# Autodesk Inventor assembly: Ensamble_general
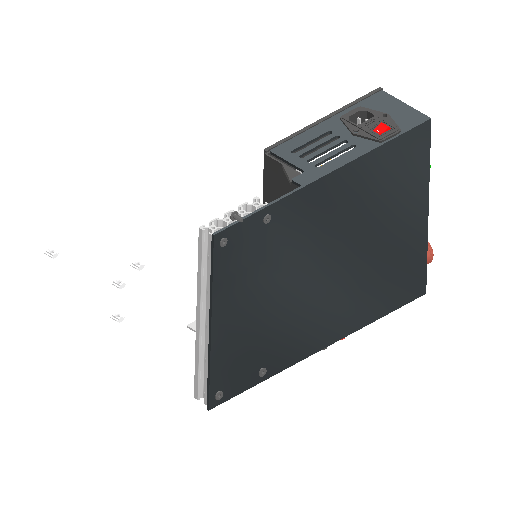
[picture p0: Inventor's stored thumbnail of the model, 512x512]
Saved by Autodesk Inventor 2025 (Build 290162000, 162)
## iProperties
Created: 2026-01-23
Part Number: Ensamble_general
Document SubType Name: Assembly
Designer: HP
Author: HP
## Documents named in this file (15)
- C:\Users\HP\Desktop\CAD\Ensamble_general.iam
- C:\Users\HP\Desktop\CAD\Chasis\Chasis_CONTROL.ipt
- C:\Users\HP\Desktop\CAD\AC_INTERUP\AC_INTERUP.ipt
- C:\Users\HP\Desktop\CAD\Banana Socket (Red)\Banana Socket (Red).ipt
- C:\Users\HP\Desktop\CAD\Banana Socket (Black)\Banana Socket (Black).ipt
- C:\Users\HP\Desktop\CAD\RED LED BULB_F\RED LED BULB_F.ipt
- C:\Users\HP\Desktop\CAD\GREEN LED BULB_F\GREEN LED BULB_F.ipt
- C:\Users\HP\Desktop\CAD\Profiles\Profiles.ipt
- C:\Users\HP\Desktop\CAD\Fuente-switching\Fuente-switching.iam
- C:\Users\HP\Desktop\CAD\E-Stop\E-Stop.ipt
- C:\Users\HP\Desktop\CAD\Tapa_chasis.ipt
- C:\Users\HP\Desktop\CAD\BRACKET_MOTOR.ipt
- C:\Users\HP\Desktop\CAD\DC Planetary Gear Brush Motor (PZ22GR9120R-084BBH)\DC Planetary Gear Brush Motor (PZ22GR9120R-084BBH).ipt
- C:\Users\HP\Desktop\CAD\Slider T-Nut for 2020 - M5\Slider T-Nut for 2020 - M5.ipt
- C:\Users\HP\Desktop\CAD\TORNILLO ALLEN CABEZA PLANA M3x0.5x6\TORNILLO ALLEN CABEZA PLANA M5x0.5x6.ipt
## Components (35 placed, 14 different names)
1. Chasis_CONTROL:1 — Coincidencia:1, Coincidencia:2, Coincidencia:3, Coincidencia:4, Coincidencia:5, Coincidencia:6, Coincidencia:7, Coincidencia:9, Coincidencia:10, Coincidencia:11, Coincidencia:12, Nivelación:1, Coincidencia:14, Nivelación:2, Coincidencia:15, Coincidencia:16, Nivelación:3, Coincidencia:19, Coincidencia:20, Coincidencia:21, Coincidencia:22, Coincidencia:23, Coincidencia:34, Coincidencia:37, Coincidencia:39, Coincidencia:41, Coincidencia:50, Coincidencia:51, Coincidencia:52, Coincidencia:53, Coincidencia:54, Coincidencia:55, Coincidencia:56, Coincidencia:57
2. AC_INTERUP:1 — Coincidencia:1, Coincidencia:2, Coincidencia:3
3. Banana Socket (Red):1 — Coincidencia:4, Coincidencia:5
4. Banana Socket (Black):1 — Coincidencia:6, Coincidencia:7
5. RED LED BULB_F:1 — Coincidencia:9, Coincidencia:12
6. GREEN LED BULB_F:1 — Coincidencia:10, Coincidencia:11
7. Profiles:1 — Nivelación:1, Coincidencia:14, Nivelación:2, Nivelación:5, Coincidencia:28, Nivelación:6, Coincidencia:32, Coincidencia:33, Coincidencia:36, Coincidencia:38, Coincidencia:40, Coincidencia:42, Coincidencia:44, Coincidencia:46, Coincidencia:48
8. Fuente-switching:1 [sub-assembly] — Coincidencia:15, Coincidencia:16, Nivelación:3
9. E-Stop:1 — Coincidencia:19, Coincidencia:20
10. Tapa_chasis:1 — Coincidencia:21, Coincidencia:22, Coincidencia:23, Coincidencia:24, Coincidencia:25, Coincidencia:26, Coincidencia:27
11. Banana Socket (Black):2 — Coincidencia:24, Coincidencia:25
12. Banana Socket (Red):2 — Coincidencia:26, Coincidencia:27
13. BRACKET_MOTOR:1 — Nivelación:5, Coincidencia:28, Nivelación:6, Coincidencia:29, Nivelación:7, Coincidencia:43, Coincidencia:45, Coincidencia:47, Coincidencia:49, Coincidencia:58, Coincidencia:59, Coincidencia:60, Coincidencia:61, Coincidencia:62, Coincidencia:63, Coincidencia:64, Coincidencia:65
14. DC Planetary Gear Brush Motor (PZ22GR9120R-084BBH):1 — Coincidencia:29, Nivelación:7
15. Slider T-Nut for 2020 - M5:1 — Coincidencia:32, Coincidencia:33, Coincidencia:34
16. Slider T-Nut for 2020 - M5:2 — Coincidencia:36, Coincidencia:37
17. Slider T-Nut for 2020 - M5:3
18. Slider T-Nut for 2020 - M5:4 — Coincidencia:42, Coincidencia:43
19. Slider T-Nut for 2020 - M5:5 — Coincidencia:48, Coincidencia:49
20. Slider T-Nut for 2020 - M5:6 — Coincidencia:38, Coincidencia:39
21. Slider T-Nut for 2020 - M5:7 — Coincidencia:40, Coincidencia:41
22. Slider T-Nut for 2020 - M5:8 — Coincidencia:44, Coincidencia:45
23. Slider T-Nut for 2020 - M5:9 — Coincidencia:46, Coincidencia:47
24. Slider T-Nut for 2020 - M5:10
25. Slider T-Nut for 2020 - M5:11
26. Slider T-Nut for 2020 - M5:12
27. TORNILLO ALLEN CABEZA PLANA M5x0.5x6:1 — Coincidencia:62, Coincidencia:63
28. TORNILLO ALLEN CABEZA PLANA M5x0.5x6:2 — Coincidencia:56, Coincidencia:57
29. TORNILLO ALLEN CABEZA PLANA M5x0.5x6:3 — Coincidencia:50, Coincidencia:51
30. TORNILLO ALLEN CABEZA PLANA M5x0.5x6:4 — Coincidencia:52, Coincidencia:53
31. TORNILLO ALLEN CABEZA PLANA M5x0.5x6:5 — Coincidencia:64, Coincidencia:65
32. TORNILLO ALLEN CABEZA PLANA M5x0.5x6:6
33. TORNILLO ALLEN CABEZA PLANA M5x0.5x6:7 — Coincidencia:60, Coincidencia:61
34. TORNILLO ALLEN CABEZA PLANA M5x0.5x6:8 — Coincidencia:58, Coincidencia:59
35. TORNILLO ALLEN CABEZA PLANA M5x0.5x6:9 — Coincidencia:54, Coincidencia:55
## Relationships (64: Mate 58, Flush 6)
- Coincidencia:1 [Mate]: Chasis_CONTROL:1 ↔ AC_INTERUP:1
- Coincidencia:2 [Mate]: Chasis_CONTROL:1 ↔ AC_INTERUP:1
- Coincidencia:3 [Mate]: Chasis_CONTROL:1 ↔ AC_INTERUP:1
- Coincidencia:4 [Mate]: Chasis_CONTROL:1 ↔ Banana Socket (Red):1
- Coincidencia:5 [Mate]: Chasis_CONTROL:1 ↔ Banana Socket (Red):1
- Coincidencia:6 [Mate]: Chasis_CONTROL:1 ↔ Banana Socket (Black):1
- Coincidencia:7 [Mate]: Chasis_CONTROL:1 ↔ Banana Socket (Black):1
- Coincidencia:9 [Mate]: Chasis_CONTROL:1 ↔ RED LED BULB_F:1
- Coincidencia:10 [Mate]: Chasis_CONTROL:1 ↔ GREEN LED BULB_F:1
- Coincidencia:11 [Mate]: Chasis_CONTROL:1 ↔ GREEN LED BULB_F:1
- Coincidencia:12 [Mate]: Chasis_CONTROL:1 ↔ RED LED BULB_F:1
- Nivelación:1 [Flush] (3 mm): Chasis_CONTROL:1 ↔ Profiles:1
- Coincidencia:14 [Mate]: Chasis_CONTROL:1 ↔ Profiles:1
- Nivelación:2 [Flush] (2 mm): Chasis_CONTROL:1 ↔ Profiles:1
- Coincidencia:15 [Mate]: Chasis_CONTROL:1 ↔ Fuente-switching:1
- Coincidencia:16 [Mate] (5 mm): Chasis_CONTROL:1 ↔ Fuente-switching:1
- Nivelación:3 [Flush] (20 mm): Chasis_CONTROL:1 ↔ Fuente-switching:1
- Coincidencia:19 [Mate]: Chasis_CONTROL:1 ↔ E-Stop:1
- Coincidencia:20 [Mate]: Chasis_CONTROL:1 ↔ E-Stop:1
- Coincidencia:21 [Mate]: Chasis_CONTROL:1 ↔ Tapa_chasis:1
- Coincidencia:22 [Mate]: Chasis_CONTROL:1 ↔ Tapa_chasis:1
- Coincidencia:23 [Mate]: Chasis_CONTROL:1 ↔ Tapa_chasis:1
- Coincidencia:24 [Mate]: Tapa_chasis:1 ↔ Banana Socket (Black):2
- Coincidencia:25 [Mate]: Tapa_chasis:1 ↔ Banana Socket (Black):2
- Coincidencia:26 [Mate]: Tapa_chasis:1 ↔ Banana Socket (Red):2
- Coincidencia:27 [Mate]: Tapa_chasis:1 ↔ Banana Socket (Red):2
- Nivelación:5 [Flush] (20 mm): Profiles:1 ↔ BRACKET_MOTOR:1
- Coincidencia:28 [Mate]: Profiles:1 ↔ BRACKET_MOTOR:1
- Nivelación:6 [Flush] (20 mm): Profiles:1 ↔ BRACKET_MOTOR:1
- Coincidencia:29 [Mate]: BRACKET_MOTOR:1 ↔ DC Planetary Gear Brush Motor (PZ22GR9120R-084BBH):1
- Nivelación:7 [Flush]: BRACKET_MOTOR:1 ↔ DC Planetary Gear Brush Motor (PZ22GR9120R-084BBH):1
- Coincidencia:32 [Mate]: Profiles:1 ↔ Slider T-Nut for 2020 - M5:1
- Coincidencia:33 [Mate]: Profiles:1 ↔ Slider T-Nut for 2020 - M5:1
- Coincidencia:34 [Mate]: Chasis_CONTROL:1 ↔ Slider T-Nut for 2020 - M5:1
- Coincidencia:36 [Mate]: Profiles:1 ↔ Slider T-Nut for 2020 - M5:2
- Coincidencia:37 [Mate]: Chasis_CONTROL:1 ↔ Slider T-Nut for 2020 - M5:2
- Coincidencia:38 [Mate]: Profiles:1 ↔ Slider T-Nut for 2020 - M5:6
- Coincidencia:39 [Mate]: Chasis_CONTROL:1 ↔ Slider T-Nut for 2020 - M5:6
- Coincidencia:40 [Mate]: Profiles:1 ↔ Slider T-Nut for 2020 - M5:7
- Coincidencia:41 [Mate]: Chasis_CONTROL:1 ↔ Slider T-Nut for 2020 - M5:7
- Coincidencia:42 [Mate]: Profiles:1 ↔ Slider T-Nut for 2020 - M5:4
- Coincidencia:43 [Mate]: BRACKET_MOTOR:1 ↔ Slider T-Nut for 2020 - M5:4
- Coincidencia:44 [Mate]: Profiles:1 ↔ Slider T-Nut for 2020 - M5:8
- Coincidencia:45 [Mate]: BRACKET_MOTOR:1 ↔ Slider T-Nut for 2020 - M5:8
- Coincidencia:46 [Mate]: Profiles:1 ↔ Slider T-Nut for 2020 - M5:9
- Coincidencia:47 [Mate]: BRACKET_MOTOR:1 ↔ Slider T-Nut for 2020 - M5:9
- Coincidencia:48 [Mate]: Profiles:1 ↔ Slider T-Nut for 2020 - M5:5
- Coincidencia:49 [Mate]: BRACKET_MOTOR:1 ↔ Slider T-Nut for 2020 - M5:5
- Coincidencia:50 [Mate] (1 mm): Chasis_CONTROL:1 ↔ TORNILLO ALLEN CABEZA PLANA M5x0.5x6:3
- Coincidencia:51 [Mate]: Chasis_CONTROL:1 ↔ TORNILLO ALLEN CABEZA PLANA M5x0.5x6:3
- Coincidencia:52 [Mate]: Chasis_CONTROL:1 ↔ TORNILLO ALLEN CABEZA PLANA M5x0.5x6:4
- Coincidencia:53 [Mate] (1 mm): Chasis_CONTROL:1 ↔ TORNILLO ALLEN CABEZA PLANA M5x0.5x6:4
- Coincidencia:54 [Mate]: Chasis_CONTROL:1 ↔ TORNILLO ALLEN CABEZA PLANA M5x0.5x6:9
- Coincidencia:55 [Mate] (1 mm): Chasis_CONTROL:1 ↔ TORNILLO ALLEN CABEZA PLANA M5x0.5x6:9
- Coincidencia:56 [Mate]: Chasis_CONTROL:1 ↔ TORNILLO ALLEN CABEZA PLANA M5x0.5x6:2
- Coincidencia:57 [Mate] (1 mm): Chasis_CONTROL:1 ↔ TORNILLO ALLEN CABEZA PLANA M5x0.5x6:2
- Coincidencia:58 [Mate]: BRACKET_MOTOR:1 ↔ TORNILLO ALLEN CABEZA PLANA M5x0.5x6:8
- Coincidencia:59 [Mate] (1 mm): BRACKET_MOTOR:1 ↔ TORNILLO ALLEN CABEZA PLANA M5x0.5x6:8
- Coincidencia:60 [Mate]: BRACKET_MOTOR:1 ↔ TORNILLO ALLEN CABEZA PLANA M5x0.5x6:7
- Coincidencia:61 [Mate] (1 mm): BRACKET_MOTOR:1 ↔ TORNILLO ALLEN CABEZA PLANA M5x0.5x6:7
- Coincidencia:62 [Mate]: BRACKET_MOTOR:1 ↔ TORNILLO ALLEN CABEZA PLANA M5x0.5x6:1
- Coincidencia:63 [Mate] (1 mm): BRACKET_MOTOR:1 ↔ TORNILLO ALLEN CABEZA PLANA M5x0.5x6:1
- Coincidencia:64 [Mate]: BRACKET_MOTOR:1 ↔ TORNILLO ALLEN CABEZA PLANA M5x0.5x6:5
- Coincidencia:65 [Mate] (1 mm): BRACKET_MOTOR:1 ↔ TORNILLO ALLEN CABEZA PLANA M5x0.5x6:5
